# Autodesk Inventor assembly: 5. asjdjasdh
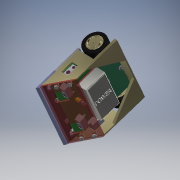
[picture p0: Inventor's stored thumbnail of the model, 180x180]
Saved by Autodesk Inventor 2017 (Build 210142000, 142)
## iProperties
Created: 2016-11-21
Part Number: 5. asjdjasdh
Document SubType Name: Assembly
Designer: Shichi
Author: Shichi
## Documents named in this file (5)
- E:\ms_lol\H3FTY\Model\5. ALL_z_Front.iam
- E:\ms_lol\H3FTY\Model\4. ALL_bez_Front.iam
- C:\Users\Shichi\Documents\Inventor\Content Center Files\R2017\en-US\AS 1112 (2)\AS 1112 - M2,5  Type 5.ipt
- C:\Users\Shichi\Documents\Inventor\Content Center Files\R2017\en-US\AS 1110\AS 1110 - M2,5 x 6.ipt
- E:\ms_lol\H3FTY\Model\Fronty\Front.ipt
## Components (10 placed, 4 different names)
1. 4. ALL_bez_Front:1 [sub-assembly] — Insert:1, Insert:2, Insert:3, Insert:4, Insert:5, Insert:6
2. AS 1110 - Metric M2,5 x 6:1 — Insert:4
3. AS 1110 - Metric M2,5 x 6:2 — Insert:3
4. AS 1110 - Metric M2,5 x 6:3 — Insert:2
5. AS 1110 - Metric M2,5 x 6:4 — Insert:1
6. Front:1 — Insert:5, Insert:6, Insert:7, Insert:8, Insert:9, Insert:10
7. AS 1112 (2) - Metric M2,5  Type 5:1 — Insert:7
8. AS 1112 (2) - Metric M2,5  Type 5:2 — Insert:9
9. AS 1112 (2) - Metric M2,5  Type 5:3 — Insert:10
10. AS 1112 (2) - Metric M2,5  Type 5:4 — Insert:8
## Relationships (10: Insert 10)
- Insert:1: 4. ALL_bez_Front:1 ↔ AS 1110 - Metric M2,5 x 6:4
- Insert:2: 4. ALL_bez_Front:1 ↔ AS 1110 - Metric M2,5 x 6:3
- Insert:3: 4. ALL_bez_Front:1 ↔ AS 1110 - Metric M2,5 x 6:2
- Insert:4: 4. ALL_bez_Front:1 ↔ AS 1110 - Metric M2,5 x 6:1
- Insert:5: 4. ALL_bez_Front:1 ↔ Front:1
- Insert:6: 4. ALL_bez_Front:1 ↔ Front:1
- Insert:7: Front:1 ↔ AS 1112 (2) - Metric M2,5  Type 5:1
- Insert:8: Front:1 ↔ AS 1112 (2) - Metric M2,5  Type 5:4
- Insert:9: Front:1 ↔ AS 1112 (2) - Metric M2,5  Type 5:2
- Insert:10: Front:1 ↔ AS 1112 (2) - Metric M2,5  Type 5:3
